# Autodesk Inventor assembly: Toaster Heating Simulation Model
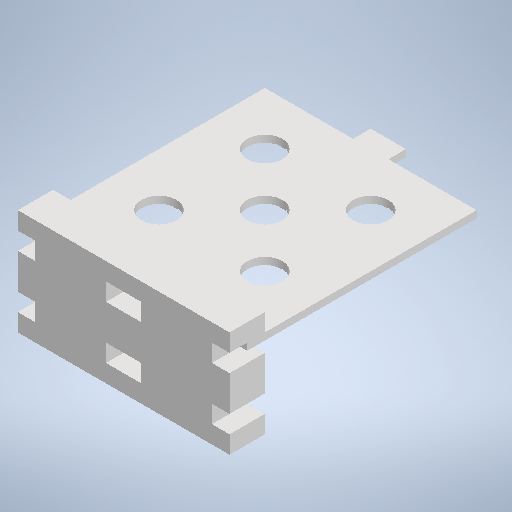
[picture p0: Inventor's stored thumbnail of the model, 512x512]
Saved by Autodesk Inventor 2025.1 (Build 291241020, 241B)
## iProperties
Created: 2024-10-29
Part Number: Toaster Heating Simulation Model
Document SubType Name: Assembly
Designer: jjk
Author: jjk
## Documents named in this file (4)
- C:\Users\jjk\Desktop\Capstone CAD\Version 2\Toaster Heating Simulation Model.iam
- C:\Users\jjk\Desktop\Capstone CAD\Version 2\Base.ipt
- C:\Users\jjk\Desktop\Capstone CAD\Version 2\Heating board.ipt
- C:\Users\jjk\Desktop\Capstone CAD\Version 2\flat 32 gauge nichrome wire.ipt
## Components (8 placed, 3 different names)
1. Base:1 — Mate:1, Mate:2, Mate:3, Flush:2, Flush:4, Flush:6, Flush:8, Flush:10, Flush:12
2. Heating board:1 — Mate:1, Mate:2, Mate:3, Mate:4, Flush:1, Flush:3, Mate:5, Flush:5, Mate:6, Flush:7, Mate:7, Flush:9, Mate:8, Flush:11, Mate:9
3. flat 32 gauge nichrome wire:2 — Mate:4, Flush:1, Flush:2
4. flat 32 gauge nichrome wire:1 — Flush:3, Mate:5, Flush:4
5. flat 32 gauge nichrome wire:3 — Flush:5, Mate:6, Flush:6
6. flat 32 gauge nichrome wire:4 — Flush:7, Mate:7, Flush:8
7. flat 32 gauge nichrome wire:5 — Flush:9, Mate:8, Flush:10
8. flat 32 gauge nichrome wire:6 — Flush:11, Mate:9, Flush:12
## Relationships (21: Flush 12, Mate 9)
- Mate:1: Base:1 ↔ Heating board:1
- Mate:2: Base:1 ↔ Heating board:1
- Mate:3: Base:1 ↔ Heating board:1
- Mate:4: Heating board:1 ↔ flat 32 gauge nichrome wire:2
- Flush:1: Heating board:1 ↔ flat 32 gauge nichrome wire:2
- Flush:2 (-139.7 mm): Base:1 ↔ flat 32 gauge nichrome wire:2
- Flush:3: Heating board:1 ↔ flat 32 gauge nichrome wire:1
- Mate:5: Heating board:1 ↔ flat 32 gauge nichrome wire:1
- Flush:4 (-127 mm): Base:1 ↔ flat 32 gauge nichrome wire:1
- Flush:5: Heating board:1 ↔ flat 32 gauge nichrome wire:3
- Mate:6: Heating board:1 ↔ flat 32 gauge nichrome wire:3
- Flush:6 (-101.6 mm): Base:1 ↔ flat 32 gauge nichrome wire:3
- Flush:7: Heating board:1 ↔ flat 32 gauge nichrome wire:4
- Mate:7: Heating board:1 ↔ flat 32 gauge nichrome wire:4
- Flush:8 (-88.9 mm): Base:1 ↔ flat 32 gauge nichrome wire:4
- Flush:9: Heating board:1 ↔ flat 32 gauge nichrome wire:5
- Mate:8: Heating board:1 ↔ flat 32 gauge nichrome wire:5
- Flush:10 (-63.5 mm): Base:1 ↔ flat 32 gauge nichrome wire:5
- Flush:11: Heating board:1 ↔ flat 32 gauge nichrome wire:6
- Mate:9: Heating board:1 ↔ flat 32 gauge nichrome wire:6
- Flush:12 (-50.8 mm): Base:1 ↔ flat 32 gauge nichrome wire:6
## Named parameters: Finish1_Area = 216.6, Finish2_Area = 216.6
note: some values were not read from the file. Shown as the stored number, unit unknown: "Finish1_Area", "Finish2_Area".
